# Autodesk Inventor assembly: компановка_платы
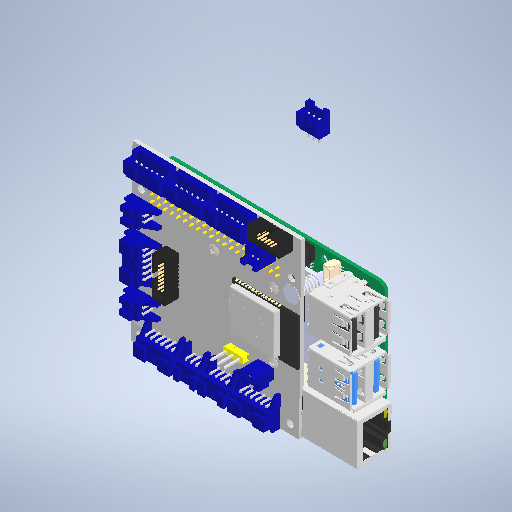
[picture p0: Inventor's stored thumbnail of the model, 512x512]
Saved by Autodesk Inventor 2025 (Build 290162000, 162)
## iProperties
Created: 2026-07-21
Part Number: компановка_платы
Document SubType Name: Assembly
Designer: garin
Author: garin
## Documents named in this file (15)
- C:\Users\garin\Documents\Git\TheseusV2_Maze\Construction\компановка_платы.iam
- C:\Users\garin\Documents\models\altium_models\idc-connectors\1.27mm\CONB127P-2R-14W_TH\CONB127P-2R-14W_TH.ipt
- C:\Users\garin\Documents\models\altium_models\ESP32-S3-WROOM\ESP32-S3-WROOM.ipt
- C:\Users\garin\Documents\models\altium_models\rpi-5b_no_graphics\rpi-5b_no_graphics.ipt
- C:\Users\garin\Documents\models\altium_models\PBD-40\PBD-40.ipt
- C:\Users\garin\Documents\Git\TheseusV2_Maze\Construction\board_rpi.ipt
- C:\Users\garin\Documents\models\altium_models\pls_connectors\PLS-3\PLS-3.ipt
- C:\Users\garin\Documents\Git\TheseusV2_Maze\Construction\Theseus_v2\Heatsink+fan RPi-5\Heatsink+fan RPi-5.ipt
- C:\Users\garin\Documents\models\altium_models\jst_pa\S02B-PASK-2\S02B-PASK-2.ipt
- C:\Users\garin\Documents\models\altium_models\jst_pa\S03B-PASK-2\S03B-PASK-2.ipt
- C:\Users\garin\Documents\models\altium_models\jst_pa\S04B-PASK-2\S04B-PASK-2.ipt
- C:\Users\garin\Documents\models\altium_models\jst_pa\S06B-PASK-2\S06B-PASK-2.ipt
- C:\Users\garin\Documents\Git\TheseusV2_Maze\Construction\Theseus_v2\B02B-PASK\B02B-PASK.ipt
- C:\Users\garin\Documents\Git\TheseusV2_Maze\Construction\Theseus_v2\B03B-PASK\B03B-PASK.ipt
- C:\Users\garin\Documents\models\altium_models\idc-connectors\1.27mm\CONB127P-2R-10W_TH\CONB127P-2R-10W_TH.ipt
## Components (21 placed, 14 different names)
1. CONB127P-2R-14W_TH:1 — Совмещение:4, Заподлицо:49
2. ESP32-S3-WROOM:1 — Совмещение:60, Заподлицо:36
3. rpi-5b_no_graphics:1 — Совмещение:1, Заподлицо:1, Заподлицо:2, Совмещение:72, Совмещение:73, Угол:1
4. PBD-40:1 — Совмещение:1, Заподлицо:1, Заподлицо:2, Совмещение:108
5. board_rpi:1 — Совмещение:4, Совмещение:60, Заподлицо:36, Совмещение:82, Совмещение:106, Заподлицо:52, Совмещение:108, Совмещение:110, Заподлицо:56, Совмещение:113, Заподлицо:58, Заподлицо:115, Совмещение:115, Заподлицо:59, Совмещение:117, Заподлицо:60, Совмещение:119, Заподлицо:116, Совмещение:121, Заподлицо:117, Совмещение:122, Совмещение:124, Заподлицо:118, Заподлицо:119, Совмещение:127, Заподлицо:120, Совмещение:129
6. Heatsink+fan RPi-5:1 — Совмещение:72, Совмещение:73, Угол:1
7. PLS-3:1 — Совмещение:82, Совмещение:126
8. S03B-PASK-2:1 — Совмещение:117, Заподлицо:60, Совмещение:118
9. S04B-PASK-2:1 — Совмещение:115, Совмещение:116, Заподлицо:59, Совмещение:118
10. S06B-PASK-2:4 — Совмещение:110, Заподлицо:56, Совмещение:123, Заподлицо:49
11. S02B-PASK-2:3 — Совмещение:119, Заподлицо:116, Совмещение:120
12. S02B-PASK-2:4 — Совмещение:121, Заподлицо:117, Совмещение:122, Совмещение:123
13. B02B-PASK:1 — Совмещение:124, Совмещение:125, Заподлицо:118, Совмещение:126
14. B03B-PASK:1
15. CONB127P-2R-10W_TH:1 — Совмещение:127, Заподлицо:120, Совмещение:128, Совмещение:130
16. B02B-PASK:2 — Совмещение:129, Совмещение:130, Совмещение:131
17. S06B-PASK-2:1 — Совмещение:106, Заподлицо:52, Совмещение:128, Совмещение:131
18. S06B-PASK-2:2
19. S06B-PASK-2:3 — Заподлицо:119
20. S06B-PASK-2:5 — Совмещение:113, Заподлицо:58, Заподлицо:115, Совмещение:116, Совмещение:125
21. S06B-PASK-2:6 — Совмещение:120
## Component patterns: (3 elements, first: S06B-PASK-2:1), (2 elements, first: S06B-PASK-2:5)
## Relationships (43: Mate 27, Flush 15, Angle 1)
- Совмещение:1 [Mate]: rpi-5b_no_graphics:1 ↔ PBD-40:1
- Заподлицо:1 [Flush]: rpi-5b_no_graphics:1 ↔ PBD-40:1
- Заподлицо:2 [Flush]: rpi-5b_no_graphics:1 ↔ PBD-40:1
- Совмещение:4 [Mate]: CONB127P-2R-14W_TH:1 ↔ board_rpi:1
- Совмещение:60 [Mate]: ESP32-S3-WROOM:1 ↔ board_rpi:1
- Заподлицо:36 [Flush]: ESP32-S3-WROOM:1 ↔ board_rpi:1
- Совмещение:72 [Mate]: rpi-5b_no_graphics:1 ↔ Heatsink+fan RPi-5:1
- Совмещение:73 [Mate]: rpi-5b_no_graphics:1 ↔ Heatsink+fan RPi-5:1
- Угол:1 [Angle] (0 deg): rpi-5b_no_graphics:1 ↔ Heatsink+fan RPi-5:1
- Совмещение:82 [Mate]: board_rpi:1 ↔ PLS-3:1
- Заподлицо:49 [Flush] (-0.595 mm): CONB127P-2R-14W_TH:1 ↔ S06B-PASK-2:4
- Совмещение:106 [Mate]: board_rpi:1 ↔ S06B-PASK-2:1
- Заподлицо:52 [Flush]: board_rpi:1 ↔ S06B-PASK-2:1
- Совмещение:108 [Mate]: PBD-40:1 ↔ board_rpi:1
- Совмещение:110 [Mate]: board_rpi:1 ↔ S06B-PASK-2:4
- Заподлицо:56 [Flush]: board_rpi:1 ↔ S06B-PASK-2:4
- Совмещение:113 [Mate]: board_rpi:1 ↔ S06B-PASK-2:5
- Заподлицо:58 [Flush]: board_rpi:1 ↔ S06B-PASK-2:5
- Заподлицо:115 [Flush] (-7.25 mm): board_rpi:1 ↔ S06B-PASK-2:5
- Совмещение:115 [Mate]: board_rpi:1 ↔ S04B-PASK-2:1
- Совмещение:116 [Mate] (1.5 mm): S04B-PASK-2:1 ↔ S06B-PASK-2:5
- Заподлицо:59 [Flush]: board_rpi:1 ↔ S04B-PASK-2:1
- Совмещение:117 [Mate]: board_rpi:1 ↔ S03B-PASK-2:1
- Заподлицо:60 [Flush]: board_rpi:1 ↔ S03B-PASK-2:1
- Совмещение:118 [Mate] (1.5 mm): S03B-PASK-2:1 ↔ S04B-PASK-2:1
- Совмещение:119 [Mate]: board_rpi:1 ↔ S02B-PASK-2:3
- Заподлицо:116 [Flush]: board_rpi:1 ↔ S02B-PASK-2:3
- Совмещение:120 [Mate] (1 mm): S02B-PASK-2:3 ↔ S06B-PASK-2:6
- Совмещение:121 [Mate]: board_rpi:1 ↔ S02B-PASK-2:4
- Заподлицо:117 [Flush]: board_rpi:1 ↔ S02B-PASK-2:4
- Совмещение:122 [Mate] (3 mm): board_rpi:1 ↔ S02B-PASK-2:4
- Совмещение:123 [Mate] (5.4 mm): S06B-PASK-2:4 ↔ S02B-PASK-2:4
- Совмещение:124 [Mate]: board_rpi:1 ↔ B02B-PASK:1
- Совмещение:125 [Mate] (2 mm): B02B-PASK:1 ↔ S06B-PASK-2:5
- Заподлицо:118 [Flush] (10 mm): board_rpi:1 ↔ B02B-PASK:1
- Совмещение:126 [Mate] (3.42 mm): PLS-3:1 ↔ B02B-PASK:1
- Заподлицо:119 [Flush] (-2.92 mm): board_rpi:1 ↔ S06B-PASK-2:3
- Совмещение:127 [Mate]: board_rpi:1 ↔ CONB127P-2R-10W_TH:1
- Заподлицо:120 [Flush]: board_rpi:1 ↔ CONB127P-2R-10W_TH:1
- Совмещение:128 [Mate] (1.5 mm): CONB127P-2R-10W_TH:1 ↔ S06B-PASK-2:1
- Совмещение:129 [Mate]: board_rpi:1 ↔ B02B-PASK:2
- Совмещение:130 [Mate] (1.5 mm): CONB127P-2R-10W_TH:1 ↔ B02B-PASK:2
- Совмещение:131 [Mate] (1.5 mm): B02B-PASK:2 ↔ S06B-PASK-2:1
